# Autodesk Inventor assembly: Partial Pull Drawer 30 kg
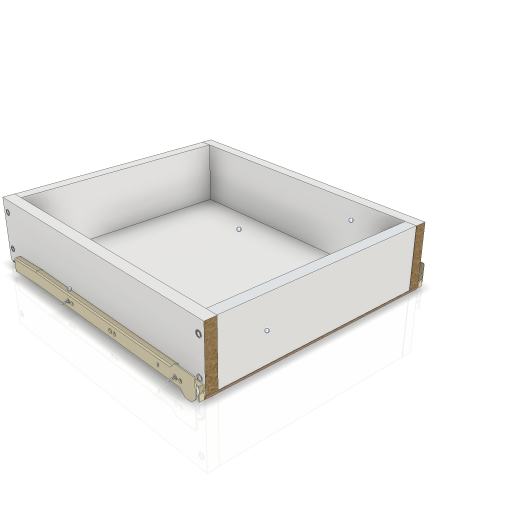
[picture p0: Inventor's stored thumbnail of the model, 512x512]
Saved by Autodesk Inventor 2024 (Build 280153000, 153)
## iProperties
Category: Drawer
RuleStatus: InUse
Created: 2015-02-10
Part Number: Partial Pull Drawer 30 kg
Document SubType Name: Assembly
Designer: SauliusD
Description: Partial Pull Drawer 30 kg
AfterAnyParamChange0: Screw Positioning and Ammount Control
AfterAnyParamChange1: Change Skeleton Parameters
Author: SauliusD
## Documents named in this file (15)
- C:\W4INV 2024 Design\iBOX LIBRARY\Drawers\Partial Pull Drawer\Partial Pull Drawer 30 kg.iam
- C:\W4INV 2024 Design\iBOX LIBRARY\Drawers\Partial Pull Drawer\Parts\Front.ipt
- C:\W4INV 2024 Design\iBOX LIBRARY\Drawers\Partial Pull Drawer\Parts\Left.ipt
- C:\W4INV 2024 Design\iBOX LIBRARY\Drawers\Partial Pull Drawer\Parts\Right.ipt
- C:\W4INV 2024 Design\iBOX LIBRARY\Drawers\Partial Pull Drawer\Parts\Back.ipt
- C:\W4INV 2024 Design\iBOX LIBRARY\Drawers\Partial Pull Drawer\Parts\Bottom.ipt
- C:\W4INV 2024 Design\iBOX LIBRARY\Drawers\Partial Pull Drawer\Parts\Right sliding Rail.ipt
- C:\W4INV 2024 Design\iBOX LIBRARY\Drawers\Partial Pull Drawer\Parts\Right fixed Rail.ipt
- C:\W4INV 2024 Design\iBOX LIBRARY\Drawers\Partial Pull Drawer\Parts\Left fixed Rail.ipt
- C:\W4INV 2024 Design\iBOX LIBRARY\Drawers\Partial Pull Drawer\Parts\Left Sliding Rail.ipt
- C:\W4INV 2024 Design\iBOX LIBRARY\Drawers\Partial Pull Drawer\Partial Pull Drawer 30 kg.ipt
- C:\W4INV 2024 Design\_LIBRARY\Fixed joints\Confirmat\CONFIRMAT\Confirmat L50 NB T18 PB T 18.ipt
- C:\W4INV 2024 Design\_LIBRARY\Fixed joints\Screws\WOOD SCREW CROSS RECESSED FLAT HEAD\Wood screw Cross Recessed Flat Head M3.5x16 H.ipt
- C:\W4INV 2024 Design\LIBRARY\Fixed joints\Screws\WOOD SCREW CROSS RECESSED FLAT HEAD.ipt
- C:\W4INV 2024 Design\LIBRARY\Fixed joints\Confirmat\CONFIRMAT.ipt
## Components (26 placed, 19 different names)
1. @Skeleton — Flush:1, Flush:2, Flush:3
2. Front:1 — Axis Plane:1, Pillar Board Side Plane:1, Axis Plane:2, Pillar Board Side Plane:2, Axis Plane:3, Axis Plane:4, Axis Plane:5, Pillar Board Side Plane:5, Axis Plane:6, Pillar Board Side Plane:6, Axis Plane:7, Axis Plane:8
3. Left:1 — Nestled Board Plane:1, Nestled Board Plane:3, Nestled Board Plane:5, Nestled Board Plane:7
4. Right:1 — Nestled Board Plane:2, Nestled Board Plane:4, Nestled Board Plane:6, Nestled Board Plane:8
5. Back:1 — Pillar Board Side Plane:3, Pillar Board Side Plane:4, Pillar Board Side Plane:7, Pillar Board Side Plane:8
6. Bottom:1
7. Right sliding Rail:1 — Insert:2, Insert:3
8. Right fixed Rail:1 — Insert:1
9. Left fixed Rail:1 — Insert:6
10. Left Sliding Rail:1 — Insert:4, Insert:5
11. Wood screw Cross Recessed Flat Head M3.5x16 H:9 — Insert:2
12. Wood screw Cross Recessed Flat Head M3.5x16 H:10 — Insert:3
13. Wood screw Cross Recessed Flat Head M3.5x16 H:11 — Insert:4
14. Wood screw Cross Recessed Flat Head M3.5x16 H:12 — Insert:5
15. Confirmat 1 — Axis Plane:1, Pillar Board Side Plane:1, Nestled Board Plane:1
16. Confirmat 2 — Axis Plane:2, Pillar Board Side Plane:2, Nestled Board Plane:2
17. Confirmat 3 — Axis Plane:3, Pillar Board Side Plane:3, Nestled Board Plane:3
18. Confirmat 4 — Axis Plane:4, Pillar Board Side Plane:4, Nestled Board Plane:4
19. Confirmat 5 — Axis Plane:5, Pillar Board Side Plane:5, Nestled Board Plane:5
20. Confirmat 6 — Axis Plane:6, Pillar Board Side Plane:6, Nestled Board Plane:6
21. Confirmat 7 — Axis Plane:7, Pillar Board Side Plane:7, Nestled Board Plane:7
22. Confirmat 8 — Axis Plane:8, Pillar Board Side Plane:8, Nestled Board Plane:8
23. Wood screw Cross Recessed Flat Head M3.5x16 H:13 — Insert:1
24. Wood screw Cross Recessed Flat Head M3.5x16 H:14
25. Wood screw Cross Recessed Flat Head M3.5x16 H:15 — Insert:6
26. Wood screw Cross Recessed Flat Head M3.5x16 H:16
## Component patterns: (2 elements, first: Wood screw Cross Recessed Flat Head M3.5x16 H:13), (2 elements, first: Wood screw Cross Recessed Flat Head M3.5x16 H:15)
## Relationships (33: Mate 16, Flush 11, Insert 6)
- Insert:1: Right fixed Rail:1 ↔ Wood screw Cross Recessed Flat Head M3.5x16 H:13
- Flush:1: @Skeleton
- Flush:2: @Skeleton
- Flush:3: @Skeleton
- Insert:2: Right sliding Rail:1 ↔ Wood screw Cross Recessed Flat Head M3.5x16 H:9
- Insert:3: Right sliding Rail:1 ↔ Wood screw Cross Recessed Flat Head M3.5x16 H:10
- Insert:4: Left Sliding Rail:1 ↔ Wood screw Cross Recessed Flat Head M3.5x16 H:11
- Insert:5: Left Sliding Rail:1 ↔ Wood screw Cross Recessed Flat Head M3.5x16 H:12
- Insert:6: Left fixed Rail:1 ↔ Wood screw Cross Recessed Flat Head M3.5x16 H:15
- Axis Plane:1 [Mate]: Front:1 ↔ Confirmat 1
- Pillar Board Side Plane:1 [Mate] (-9 mm): Front:1 ↔ Confirmat 1
- Nestled Board Plane:1 [Flush]: Left:1 ↔ Confirmat 1
- Axis Plane:2 [Mate]: Front:1 ↔ Confirmat 2
- Pillar Board Side Plane:2 [Mate] (-9 mm): Front:1 ↔ Confirmat 2
- Nestled Board Plane:2 [Flush]: Right:1 ↔ Confirmat 2
- Axis Plane:3 [Mate]: Front:1 ↔ Confirmat 3
- Pillar Board Side Plane:3 [Mate] (-9 mm): Back:1 ↔ Confirmat 3
- Nestled Board Plane:3 [Flush]: Left:1 ↔ Confirmat 3
- Axis Plane:4 [Mate]: Front:1 ↔ Confirmat 4
- Pillar Board Side Plane:4 [Mate] (-9 mm): Back:1 ↔ Confirmat 4
- Nestled Board Plane:4 [Flush]: Right:1 ↔ Confirmat 4
- Axis Plane:5 [Mate]: Front:1 ↔ Confirmat 5
- Pillar Board Side Plane:5 [Mate] (-9 mm): Front:1 ↔ Confirmat 5
- Nestled Board Plane:5 [Flush]: Left:1 ↔ Confirmat 5
- Axis Plane:6 [Mate]: Front:1 ↔ Confirmat 6
- Pillar Board Side Plane:6 [Mate] (-9 mm): Front:1 ↔ Confirmat 6
- Nestled Board Plane:6 [Flush]: Right:1 ↔ Confirmat 6
- Axis Plane:7 [Mate]: Front:1 ↔ Confirmat 7
- Pillar Board Side Plane:7 [Mate] (-9 mm): Back:1 ↔ Confirmat 7
- Nestled Board Plane:7 [Flush]: Left:1 ↔ Confirmat 7
- Axis Plane:8 [Mate]: Front:1 ↔ Confirmat 8
- Pillar Board Side Plane:8 [Mate] (-9 mm): Back:1 ↔ Confirmat 8
- Nestled Board Plane:8 [Flush]: Right:1 ↔ Confirmat 8
## Named parameters: Back_Screw_Position = 224 mm, Rear_Space = 10 mm, Facade_Inlet = 0 mm, Board_Thickness = 18 mm, Distance_from_bottom = 0 mm
